# Autodesk Inventor assembly: RelayCaseAssy
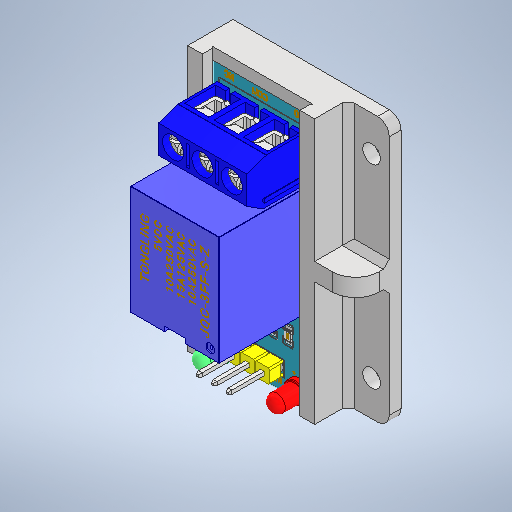
[picture p0: Inventor's stored thumbnail of the model, 512x512]
Saved by Autodesk Inventor 2025.1 (Build 291241000, 241)
## iProperties
Created: 2026-05-31
Part Number: RelayCaseAssy
Document SubType Name: Assembly
Designer: User
Author: User
## Documents named in this file (3)
- D:\One Drive\OneDrive - Politeknik Sultan Salahuddin Abdul Aziz Shah\Documents\Inventor\RobosotPSA\RelayCaseAssy.iam
- D:\One Drive\OneDrive - Politeknik Sultan Salahuddin Abdul Aziz Shah\Documents\Inventor\RobosotPSA\Relay_Module_1ch v3\Relay_Module_1ch v3\Relay_Module_1ch v3.ipt
- D:\One Drive\OneDrive - Politeknik Sultan Salahuddin Abdul Aziz Shah\Documents\Inventor\RobosotPSA\relay_case.ipt
## Components (2 placed, 2 different names)
1. Relay_Module_1ch v3:1 — Flush:1
2. relay_case:1 — Flush:1
## Relationships (1: Flush 1)
- Flush:1: Relay_Module_1ch v3:1 ↔ relay_case:1
